# Autodesk Inventor assembly: Robot
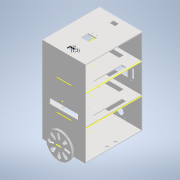
[picture p0: Inventor's stored thumbnail of the model, 180x180]
Saved by Autodesk Inventor 2020 (Build 240168000, 168)
## iProperties
Created: 2020-01-22
Part Number: Robot
Document SubType Name: Assembly
Designer: jelte
Mass: 570.337 g
Surface Area: 4038.22 cm^2
Volume: 570.337 cm^3
Density: 1 g/cm^3
Author: jelte
## Documents named in this file (8)
- E:\GIP\EA\3D Tekeningen\Versie 1\Robot.iam
- E:\GIP\EA\3D Tekeningen\Versie 1\MuurL.ipt
- E:\GIP\EA\3D Tekeningen\Versie 1\Level1 (motoren).ipt
- E:\GIP\EA\3D Tekeningen\Versie 1\Level2 (arduino).ipt
- E:\GIP\EA\3D Tekeningen\Versie 1\Level3 (voeding).ipt
- E:\GIP\EA\3D Tekeningen\Versie 1\Level4 (sensor + schakelaar).ipt
- E:\GIP\EA\3D Tekeningen\Versie 1\MuurR.ipt
- E:\GIP\EA\3D Tekeningen\Versie 3\Wiel.ipt
## Components (7 placed, 7 different names)
1. Level2 (arduino):1
2. Level3 (voeding):1
3. Level1 (motoren):1
4. Level4 (sensor + schakelaar):1 — Rigid:8, Rigid:9
5. MuurR:1 — Rigid:8, Rotational:1
6. MuurL:1 — Rigid:9
7. Wiel:1 — Rotational:1
## Relationships (3: WeldJoint 2, RevoluteJoint 1)
- Rigid:8 [WeldJoint]: Level4 (sensor + schakelaar):1 ↔ MuurR:1
- Rigid:9 [WeldJoint]: Level4 (sensor + schakelaar):1 ↔ MuurL:1
- Rotational:1 [RevoluteJoint]: MuurR:1 ↔ Wiel:1
